# Autodesk Inventor assembly: FrontPlate
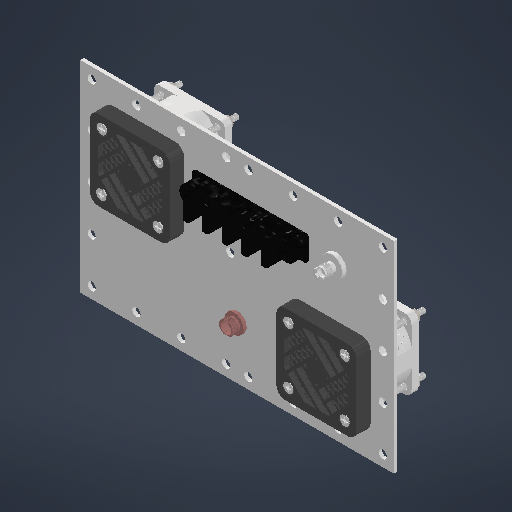
[picture p0: Inventor's stored thumbnail of the model, 512x512]
Saved by Autodesk Inventor 2026.2 (Build 302298010, 298A)
## iProperties
Created: 2026-07-30
Part Number: FrontPlate
Document SubType Name: Assembly
Designer: sonata
Author: sonata
## Documents named in this file (11)
- Z:\crush\NRDZ-Sensor_2026\Parts\FrontPlate.iam
- Z:\crush\NRDZ-Sensor_2026\Parts\NRDZ_Fan_plate\NRDZ_Fan_plate.ipt
- Z:\crush\NRDZ-Sensor_2026\Parts\Kemvent40\3D\Kemvent40\Kemvent40\Kemvent40.ipt
- Z:\crush\NRDZ-Sensor_2026\Parts\PE9134NH\PE9184NH_3D\PE9184NH_3D\PE9184NH_3D.ipt
- Z:\crush\NRDZ-Sensor_2026\Parts\52160004A.ipt
- Z:\crush\NRDZ-Sensor_2026\Parts\FOA-FCAM1-MC0D-SMH_3D\FOA-FCAM1-MC0D-SMH_3D\FOA-FCAM1-MC0D-SMH_3D.ipt
- Z:\crush\NRDZ-Sensor_2026\Parts\259-PF40281B2-1000U-A9H-ND\259-PF40281B2-1000U-A9H-ND\259-PF40281B2-1000U-A9H-ND.ipt
- Z:\crush\NRDZ-Sensor_2026\Parts\259-GF40282B1-1000U-ADP-ND\259-GF40282B1-1000U-ADP-ND\259-GF40282B1-1000U-ADP-ND.ipt
- Z:\crush\NRDZ-Sensor_2026\Parts\91420A138\91420A138_Steel Phillips Flat Head Screws\91420A138_Steel Phillips Flat Head Screws\91420A138_Steel Phillips Flat Head Screws.ipt
- Z:\crush\NRDZ-Sensor_2026\Parts\04M030050HNDIN34814\3D\04M030050HNDIN34814\04M030050HNDIN34814\04M030050HNDIN34814.ipt
- Z:\crush\NRDZ-Sensor_2026\Parts\92005A116\92005A116_Steel Pan Head Phillips Screw\92005A116_Steel Pan Head Phillips Screw\92005A116_Steel Pan Head Phillips Screw.ipt
## Components (26 placed, 10 different names)
1. NRDZ_Fan_plate:1 — Insert:1, Insert:2, Insert:3, Angle:1, Insert:4, Insert:5, Angle:2, Insert:6, Insert:7, Angle:3, Insert:8, Angle:4, Insert:25, Insert:26
2. Kemvent40:1 — Insert:2, Insert:3, Insert:9, Insert:10, Insert:11, Insert:12
3. Kemvent40:2 — Insert:1, Insert:13, Insert:14, Insert:15, Insert:16
4. PE9184NH_3D:1 — Angle:1, Insert:4
5. 52160004A:1 — Insert:5, Angle:2
6. FOA-FCAM1-MC0D-SMH_3D:1 — Insert:6
7. 259-PF40281B2-1000U-A9H-ND:1 — Insert:7, Angle:3, Insert:21, Insert:22, Insert:23, Insert:24
8. 259-GF40282B1-1000U-ADP-ND:1 — Insert:8, Angle:4, Insert:17, Insert:18, Insert:19, Insert:20
9. 04M030050HNDIN34814:1 — Insert:20
10. 04M030050HNDIN34814:2 — Insert:18
11. 04M030050HNDIN34814:3 — Insert:17
12. 04M030050HNDIN34814:4 — Insert:19
13. 04M030050HNDIN34814:5 — Insert:21
14. 04M030050HNDIN34814:6 — Insert:22
15. 04M030050HNDIN34814:8 — Insert:23
16. 04M030050HNDIN34814:7 — Insert:24
17. 92005A116_Steel Pan Head Phillips Screw:1 — Insert:25
18. 04M030050HNDIN34814:9 — Insert:26
19. 91420A138_Steel Phillips Flat Head Screws:8 — Insert:14
20. 91420A138_Steel Phillips Flat Head Screws:7 — Insert:13
21. 91420A138_Steel Phillips Flat Head Screws:6 — Insert:15
22. 91420A138_Steel Phillips Flat Head Screws:5 — Insert:16
23. 91420A138_Steel Phillips Flat Head Screws:4 — Insert:10
24. 91420A138_Steel Phillips Flat Head Screws:3 — Insert:11
25. 91420A138_Steel Phillips Flat Head Screws:2 — Insert:12
26. 91420A138_Steel Phillips Flat Head Screws:1 — Insert:9
## Relationships (30: Insert 26, Angle 4)
- Insert:1 (-8.001 mm): NRDZ_Fan_plate:1 ↔ Kemvent40:2
- Insert:2 (-8.001 mm): NRDZ_Fan_plate:1 ↔ Kemvent40:1
- Insert:3 (-8.001 mm): NRDZ_Fan_plate:1 ↔ Kemvent40:1
- Angle:1 (180 deg): NRDZ_Fan_plate:1 ↔ PE9184NH_3D:1
- Insert:4: NRDZ_Fan_plate:1 ↔ PE9184NH_3D:1
- Insert:5: NRDZ_Fan_plate:1 ↔ 52160004A:1
- Angle:2 (0 deg): NRDZ_Fan_plate:1 ↔ 52160004A:1
- Insert:6: NRDZ_Fan_plate:1 ↔ FOA-FCAM1-MC0D-SMH_3D:1
- Insert:7: NRDZ_Fan_plate:1 ↔ 259-PF40281B2-1000U-A9H-ND:1
- Angle:3 (0 deg): NRDZ_Fan_plate:1 ↔ 259-PF40281B2-1000U-A9H-ND:1
- Insert:8: NRDZ_Fan_plate:1 ↔ 259-GF40282B1-1000U-ADP-ND:1
- Angle:4 (0 deg): NRDZ_Fan_plate:1 ↔ 259-GF40282B1-1000U-ADP-ND:1
- Insert:9: Kemvent40:1 ↔ 91420A138_Steel Phillips Flat Head Screws:1
- Insert:10: Kemvent40:1 ↔ 91420A138_Steel Phillips Flat Head Screws:4
- Insert:11: Kemvent40:1 ↔ 91420A138_Steel Phillips Flat Head Screws:3
- Insert:12: Kemvent40:1 ↔ 91420A138_Steel Phillips Flat Head Screws:2
- Insert:13: Kemvent40:2 ↔ 91420A138_Steel Phillips Flat Head Screws:7
- Insert:14: Kemvent40:2 ↔ 91420A138_Steel Phillips Flat Head Screws:8
- Insert:15: Kemvent40:2 ↔ 91420A138_Steel Phillips Flat Head Screws:6
- Insert:16: Kemvent40:2 ↔ 91420A138_Steel Phillips Flat Head Screws:5
- Insert:17: 259-GF40282B1-1000U-ADP-ND:1 ↔ 04M030050HNDIN34814:3
- Insert:18: 259-GF40282B1-1000U-ADP-ND:1 ↔ 04M030050HNDIN34814:2
- Insert:19: 259-GF40282B1-1000U-ADP-ND:1 ↔ 04M030050HNDIN34814:4
- Insert:20: 259-GF40282B1-1000U-ADP-ND:1 ↔ 04M030050HNDIN34814:1
- Insert:21: 259-PF40281B2-1000U-A9H-ND:1 ↔ 04M030050HNDIN34814:5
- Insert:22: 259-PF40281B2-1000U-A9H-ND:1 ↔ 04M030050HNDIN34814:6
- Insert:23: 259-PF40281B2-1000U-A9H-ND:1 ↔ 04M030050HNDIN34814:8
- Insert:24: 259-PF40281B2-1000U-A9H-ND:1 ↔ 04M030050HNDIN34814:7
- Insert:25: NRDZ_Fan_plate:1 ↔ 92005A116_Steel Pan Head Phillips Screw:1
- Insert:26: NRDZ_Fan_plate:1 ↔ 04M030050HNDIN34814:9
